# Autodesk Inventor assembly: BallBot
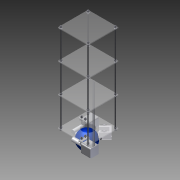
[picture p0: Inventor's stored thumbnail of the model, 180x180]
Saved by Autodesk Inventor 2012 (Build 160160000, 160)
## iProperties
Created: 2012-10-02
Part Number: BallBot
Document SubType Name: Assembly
Designer: agmlego
Author: agmlego
## Documents named in this file (16)
- H:\My Documents\Projects\BallBot\micro\CAD\BallBot.iam
- H:\My Documents\Projects\BallBot\micro\CAD\Platform.ipt
- H:\My Documents\Projects\BallBot\micro\CAD\Rod.ipt
- H:\My Documents\Projects\BallBot\micro\CAD\Ball.ipt
- \\derp\hdrives\agmeyer\My Documents\Inventor\Content Center Files\R2012\en-US\ANSI B 18.2.4.1 M(1)\ANSI B 18.2.4.1 M - M3 x 0.5Style 1.ipt
- H:\My Documents\Projects\BallBot\micro\CAD\211-13-01.ipt
- H:\My Documents\Projects\BallBot\micro\CAD\Roller.ipt
- \\derp\hdrives\agmeyer\My Documents\Inventor\Content Center Files\R2012\en-US\ANSI B18.3(08)\ANSI B18.3 - 4-48 UNF - 0.125(24).ipt
- H:\My Documents\Projects\BallBot\micro\CAD\Bottom_Platform.ipt
- H:\My Documents\Projects\BallBot\micro\CAD\Stepper_Bracket.ipt
- H:\My Documents\Projects\BallBot\micro\CAD\Tension_Housing.ipt
- H:\My Documents\Projects\BallBot\micro\CAD\Idler.ipt
- \\derp\hdrives\agmeyer\My Documents\Inventor\Content Center Files\R2012\en-US\ANSI B18.3.1M(6)\ANSI B18.3.1M - M3x0.5 x 35(1).ipt
- \\derp\hdrives\agmeyer\My Documents\Inventor\Content Center Files\R2012\en-US\ANSI B18.3.1M(6)\ANSI B18.3.1M - M2.5x0.45 x 10(1).ipt
- \\derp\hdrives\agmeyer\My Documents\Inventor\Content Center Files\R2012\en-US\ANSI B18.3.1M(6)\ANSI B18.3.1M - M3x0.5 x 10(1).ipt
- \\derp\hdrives\agmeyer\My Documents\Inventor\Content Center Files\R2012\en-US\ANSI B18.22 M\ANSI B18.22M - 3 N.ipt
## Components (103 placed, 15 different names)
1. Rod:1 — Mate:4, Mate:5, Mate:6, Mate:7, Mate:8, Mate:9, Mate:10, Mate:11, Mate:34, Mate:38, Mate:42, Mate:115, Mate:133, Mate:134, Mate:135, Mate:136, Mate:137, Mate:138, Mate:139, Mate:140, Flush:6, Flush:9
2. Rod:2 — Mate:1, Mate:3, Mate:12, Mate:13, Mate:14, Mate:15, Mate:16, Mate:17, Mate:35, Mate:39, Mate:43, Mate:114, Mate:145, Mate:146, Mate:147, Mate:148, Mate:149, Mate:150, Mate:153, Mate:154, Flush:5, Flush:11
3. Rod:3 — Mate:18, Mate:19, Mate:20, Mate:21, Mate:22, Mate:23, Mate:24, Mate:25, Mate:36, Mate:40, Mate:44, Mate:90, Mate:116, Mate:124, Mate:126, Mate:127, Mate:128, Mate:129, Mate:130, Mate:131, Mate:132, Flush:8, Flush:12
4. Rod:4 — Mate:26, Mate:27, Mate:28, Mate:29, Mate:30, Mate:31, Mate:32, Mate:33, Mate:37, Mate:41, Mate:45, Mate:117, Mate:155, Mate:156, Mate:157, Mate:158, Mate:159, Mate:160, Mate:161, Mate:162, Flush:7, Flush:10
5. Ball:1 — Tangent:5, Tangent:6, Tangent:8
6. Tension_Housing:1 — Mate:105, Mate:107, Mate:108, Mate:109, Insert:3, Insert:4
7. Idler:1 — Mate:107, Mate:108, Tangent:8
8. Forged Socket Head Cap Screw - Metric M3x0.5 x 35:1 — Insert:3
9. Hex Nut Metric M3 x 0.5:65 — Insert:4
10. 211-13-01:3 — Insert:2, Tangent:1, Tangent:2, Mate:97, Mate:98, Mate:99
11. Roller:1 — Insert:2, Mate:91, Mate:92, Tangent:6
12. Hexagon Socket Set Screw - Flat Point - Inch 4-48 UNF x 0.125:5 — Mate:91, Tangent:1
13. Hexagon Socket Set Screw - Flat Point - Inch 4-48 UNF x 0.125:7 — Mate:92, Tangent:2
14. Stepper_Bracket:1 — Mate:97, Mate:98, Mate:99, Mate:104, Insert:7, Insert:8, Mate:112, Mate:113, Insert:11, Insert:12
15. Forged Socket Head Cap Screw - Metric M2.5x0.45 x 10:3 — Insert:7
16. Forged Socket Head Cap Screw - Metric M2.5x0.45 x 10:4 — Insert:8
17. Forged Socket Head Cap Screw - Metric M3x0.5 x 10:2 — Insert:11, Mate:142
18. Forged Socket Head Cap Screw - Metric M3x0.5 x 10:4 — Insert:12, Mate:141
19. Hex Nut Metric M3 x 0.5:68 — Insert:21
20. Hex Nut Metric M3 x 0.5:69 — Insert:22
21. Plain Washer (Metric) 3 N:9 — Mate:141, Mate:227, Insert:22
22. Plain Washer (Metric) 3 N:10 — Mate:142, Mate:226, Insert:21
23. Stepper_Bracket:2 — Mate:100, Mate:101, Mate:102, Mate:103, Insert:5, Insert:6, Mate:110, Mate:111, Insert:9, Insert:10
24. 211-13-01:1 — Insert:1, Tangent:3, Tangent:4, Mate:100, Mate:101, Mate:102
25. Roller:2 — Insert:1, Mate:93, Mate:94, Tangent:5
26. Hexagon Socket Set Screw - Flat Point - Inch 4-48 UNF x 0.125:6 — Mate:94, Tangent:4
27. Hexagon Socket Set Screw - Flat Point - Inch 4-48 UNF x 0.125:8 — Mate:93, Tangent:3
28. Forged Socket Head Cap Screw - Metric M2.5x0.45 x 10:1 — Insert:5
29. Forged Socket Head Cap Screw - Metric M2.5x0.45 x 10:2 — Insert:6
30. Forged Socket Head Cap Screw - Metric M3x0.5 x 10:1 — Insert:9, Mate:143
31. Forged Socket Head Cap Screw - Metric M3x0.5 x 10:3 — Insert:10, Mate:144
32. Hex Nut Metric M3 x 0.5:66 — Insert:23
33. Hex Nut Metric M3 x 0.5:67 — Insert:24
34. Plain Washer (Metric) 3 N:11 — Mate:144, Mate:229, Insert:24
35. Plain Washer (Metric) 3 N:12 — Mate:143, Mate:228, Insert:23
36. Platform:3 — Mate:38, Mate:39, Mate:40, Mate:41, Mate:43, Mate:44, Mate:45, Mate:88, Mate:164, Mate:165, Mate:167, Mate:169, Mate:171, Mate:173, Mate:175, Mate:177
37. Hex Nut Metric M3 x 0.5:38 — Mate:31, Mate:172, Flush:7
38. Hex Nut Metric M3 x 0.5:40 — Mate:33, Mate:174
39. Hex Nut Metric M3 x 0.5:46 — Mate:9, Mate:170
40. Hex Nut Metric M3 x 0.5:47 — Mate:10, Mate:168, Flush:6
41. Hex Nut Metric M3 x 0.5:51 — Mate:12, Mate:166
42. Hex Nut Metric M3 x 0.5:56 — Mate:17, Mate:163, Flush:5
43. Hex Nut Metric M3 x 0.5:62 — Mate:23, Mate:176, Flush:8
44. Hex Nut Metric M3 x 0.5:63 — Mate:24, Mate:178
45. Plain Washer (Metric) 3 N:1 — Mate:132, Mate:177, Mate:178
46. Plain Washer (Metric) 3 N:2 — Mate:131, Mate:175, Mate:176
47. Plain Washer (Metric) 3 N:27 — Mate:133, Mate:167, Mate:168
48. Plain Washer (Metric) 3 N:28 — Mate:134, Mate:169, Mate:170
49. Plain Washer (Metric) 3 N:29 — Mate:153, Mate:163, Mate:164
50. Plain Washer (Metric) 3 N:30 — Mate:154, Mate:165, Mate:166
51. Plain Washer (Metric) 3 N:31 — Mate:155, Mate:171, Mate:172
52. Plain Washer (Metric) 3 N:32 — Mate:156, Mate:173, Mate:174
53. Platform:4 — Mate:42, Mate:88, Mate:89, Mate:90, Mate:180, Mate:181, Mate:184, Mate:185, Mate:188, Mate:189, Mate:192, Mate:193
54. Hex Nut Metric M3 x 0.5:35 — Mate:28, Mate:182
55. Hex Nut Metric M3 x 0.5:39 — Mate:32, Mate:179
56. Hex Nut Metric M3 x 0.5:41 — Mate:4, Mate:190
57. Hex Nut Metric M3 x 0.5:45 — Mate:8, Mate:187
58. Hex Nut Metric M3 x 0.5:53 — Mate:14, Mate:194
59. Hex Nut Metric M3 x 0.5:54 — Mate:15, Mate:191
60. Hex Nut Metric M3 x 0.5:60 — Mate:21, Mate:183
61. Hex Nut Metric M3 x 0.5:64 — Mate:25, Mate:186
62. Plain Washer (Metric) 3 N:3 — Mate:130, Mate:185, Mate:186
63. Plain Washer (Metric) 3 N:4 — Mate:129, Mate:183, Mate:184
64. Plain Washer (Metric) 3 N:21 — Mate:135, Mate:187, Mate:188
65. Plain Washer (Metric) 3 N:22 — Mate:136, Mate:189, Mate:190
66. Plain Washer (Metric) 3 N:23 — Mate:150, Mate:193, Mate:194
67. Plain Washer (Metric) 3 N:24 — Mate:149, Mate:191, Mate:192
68. Plain Washer (Metric) 3 N:33 — Mate:157, Mate:181, Mate:182
69. Plain Washer (Metric) 3 N:34 — Mate:158, Mate:179, Mate:180
70. Platform:2 — Mate:34, Mate:35, Mate:36, Mate:37, Mate:89, Mate:196, Mate:197, Mate:200, Mate:201, Mate:203, Mate:205, Mate:208, Mate:209
71. Hex Nut Metric M3 x 0.5:36 — Mate:29, Mate:210
72. Hex Nut Metric M3 x 0.5:37 — Mate:30, Mate:207
73. Hex Nut Metric M3 x 0.5:42 — Mate:5, Mate:199
74. Hex Nut Metric M3 x 0.5:48 — Mate:11, Mate:202
75. Hex Nut Metric M3 x 0.5:52 — Mate:13, Mate:198
76. Hex Nut Metric M3 x 0.5:55 — Mate:16, Mate:195
77. Hex Nut Metric M3 x 0.5:58 — Mate:19, Mate:206
78. Hex Nut Metric M3 x 0.5:59 — Mate:20, Mate:204
79. Plain Washer (Metric) 3 N:5 — Mate:128, Mate:205, Mate:206
80. Plain Washer (Metric) 3 N:6 — Mate:127, Mate:203, Mate:204
81. Plain Washer (Metric) 3 N:17 — Mate:147, Mate:197, Mate:198
82. Plain Washer (Metric) 3 N:18 — Mate:146, Mate:195, Mate:196
83. Plain Washer (Metric) 3 N:19 — Mate:137, Mate:199, Mate:200
84. Plain Washer (Metric) 3 N:20 — Mate:138, Mate:201, Mate:202
85. Plain Washer (Metric) 3 N:35 — Mate:159, Mate:209, Mate:210
86. Plain Washer (Metric) 3 N:36 — Mate:160, Mate:207, Mate:208
87. Bottom_Platform:1 — Mate:103, Mate:104, Mate:105, Mate:109, Mate:110, Mate:111, Mate:112, Mate:113, Mate:114, Mate:115, Mate:116, Mate:117, Mate:125, Mate:212, Mate:213, Mate:215, Mate:219, Mate:220, Mate:223, Mate:224, Mate:226, Mate:227, Mate:228, Mate:229
88. Hex Nut Metric M3 x 0.5:33 — Mate:26, Mate:214, Flush:10
89. Hex Nut Metric M3 x 0.5:34 — Mate:27, Mate:211
90. Hex Nut Metric M3 x 0.5:43 — Mate:6, Mate:225, Flush:9
91. Hex Nut Metric M3 x 0.5:44 — Mate:7, Mate:222
92. Hex Nut Metric M3 x 0.5:49 — Mate:1, Mate:221, Flush:11
93. Hex Nut Metric M3 x 0.5:50 — Mate:3, Mate:218
94. Hex Nut Metric M3 x 0.5:57 — Mate:18, Mate:216
95. Hex Nut Metric M3 x 0.5:61 — Mate:22, Mate:217, Flush:12
96. Plain Washer (Metric) 3 N:7 — Mate:126, Mate:215, Mate:216
97. Plain Washer (Metric) 3 N:8 — Mate:124, Mate:125, Mate:217
98. Plain Washer (Metric) 3 N:13 — Mate:148, Mate:218, Mate:219
99. Plain Washer (Metric) 3 N:14 — Mate:145, Mate:220, Mate:221
100. Plain Washer (Metric) 3 N:15 — Mate:139, Mate:222, Mate:223
101. Plain Washer (Metric) 3 N:16 — Mate:140, Mate:224, Mate:225
102. Plain Washer (Metric) 3 N:37 — Mate:161, Mate:211, Mate:212
103. Plain Washer (Metric) 3 N:38 — Mate:162, Mate:213, Mate:214
## Relationships (206: Mate 175, Insert 16, Flush 8, Tangent 7)
- Mate:1: Rod:2 ↔ Hex Nut Metric M3 x 0.5:49
- Mate:3: Rod:2 ↔ Hex Nut Metric M3 x 0.5:50
- Mate:4: Rod:1 ↔ Hex Nut Metric M3 x 0.5:41
- Mate:5: Rod:1 ↔ Hex Nut Metric M3 x 0.5:42
- Mate:6: Rod:1 ↔ Hex Nut Metric M3 x 0.5:43
- Mate:7: Rod:1 ↔ Hex Nut Metric M3 x 0.5:44
- Mate:8: Rod:1 ↔ Hex Nut Metric M3 x 0.5:45
- Mate:9: Rod:1 ↔ Hex Nut Metric M3 x 0.5:46
- Mate:10: Rod:1 ↔ Hex Nut Metric M3 x 0.5:47
- Mate:11: Rod:1 ↔ Hex Nut Metric M3 x 0.5:48
- Mate:12: Rod:2 ↔ Hex Nut Metric M3 x 0.5:51
- Mate:13: Rod:2 ↔ Hex Nut Metric M3 x 0.5:52
- Mate:14: Rod:2 ↔ Hex Nut Metric M3 x 0.5:53
- Mate:15: Rod:2 ↔ Hex Nut Metric M3 x 0.5:54
- Mate:16: Rod:2 ↔ Hex Nut Metric M3 x 0.5:55
- Mate:17: Rod:2 ↔ Hex Nut Metric M3 x 0.5:56
- Mate:18: Rod:3 ↔ Hex Nut Metric M3 x 0.5:57
- Mate:19: Rod:3 ↔ Hex Nut Metric M3 x 0.5:58
- Mate:20: Rod:3 ↔ Hex Nut Metric M3 x 0.5:59
- Mate:21: Rod:3 ↔ Hex Nut Metric M3 x 0.5:60
- Mate:22: Rod:3 ↔ Hex Nut Metric M3 x 0.5:61
- Mate:23: Rod:3 ↔ Hex Nut Metric M3 x 0.5:62
- Mate:24: Rod:3 ↔ Hex Nut Metric M3 x 0.5:63
- Mate:25: Rod:3 ↔ Hex Nut Metric M3 x 0.5:64
- Mate:26: Rod:4 ↔ Hex Nut Metric M3 x 0.5:33
- Mate:27: Rod:4 ↔ Hex Nut Metric M3 x 0.5:34
- Mate:28: Rod:4 ↔ Hex Nut Metric M3 x 0.5:35
- Mate:29: Rod:4 ↔ Hex Nut Metric M3 x 0.5:36
- Mate:30: Rod:4 ↔ Hex Nut Metric M3 x 0.5:37
- Mate:31: Rod:4 ↔ Hex Nut Metric M3 x 0.5:38
- Mate:32: Rod:4 ↔ Hex Nut Metric M3 x 0.5:39
- Mate:33: Rod:4 ↔ Hex Nut Metric M3 x 0.5:40
- Mate:34: Rod:1 ↔ Platform:2
- Mate:35: Rod:2 ↔ Platform:2
- Mate:36: Rod:3 ↔ Platform:2
- Mate:37: Rod:4 ↔ Platform:2
- Mate:38: Rod:1 ↔ Platform:3
- Mate:39: Rod:2 ↔ Platform:3
- Mate:40: Rod:3 ↔ Platform:3
- Mate:41: Rod:4 ↔ Platform:3
- Mate:42: Rod:1 ↔ Platform:4
- Mate:43: Rod:2 ↔ Platform:3
- Mate:44: Rod:3 ↔ Platform:3
- Mate:45: Rod:4 ↔ Platform:3
- Mate:88 (93.1 mm): Platform:3 ↔ Platform:4
- Mate:89 (93.1 mm): Platform:4 ↔ Platform:2
- Mate:90: Rod:3 ↔ Platform:4
- Insert:1: 211-13-01:1 ↔ Roller:2
- Insert:2: 211-13-01:3 ↔ Roller:1
- Mate:91: Roller:1 ↔ Hexagon Socket Set Screw - Flat Point - Inch 4-48 UNF x 0.125:5
- Mate:92: Roller:1 ↔ Hexagon Socket Set Screw - Flat Point - Inch 4-48 UNF x 0.125:7
- Mate:93: Roller:2 ↔ Hexagon Socket Set Screw - Flat Point - Inch 4-48 UNF x 0.125:8
- Mate:94: Roller:2 ↔ Hexagon Socket Set Screw - Flat Point - Inch 4-48 UNF x 0.125:6
- Tangent:1: 211-13-01:3 ↔ Hexagon Socket Set Screw - Flat Point - Inch 4-48 UNF x 0.125:5
- Tangent:2: 211-13-01:3 ↔ Hexagon Socket Set Screw - Flat Point - Inch 4-48 UNF x 0.125:7
- Tangent:3: 211-13-01:1 ↔ Hexagon Socket Set Screw - Flat Point - Inch 4-48 UNF x 0.125:8
- Tangent:4: 211-13-01:1 ↔ Hexagon Socket Set Screw - Flat Point - Inch 4-48 UNF x 0.125:6
- Tangent:5: Ball:1 ↔ Roller:2
- Tangent:6: Ball:1 ↔ Roller:1
- Mate:97: 211-13-01:3 ↔ Stepper_Bracket:1
- Mate:98: 211-13-01:3 ↔ Stepper_Bracket:1
- Mate:99: 211-13-01:3 ↔ Stepper_Bracket:1
- Mate:100: Stepper_Bracket:2 ↔ 211-13-01:1
- Mate:101: Stepper_Bracket:2 ↔ 211-13-01:1
- Mate:102: Stepper_Bracket:2 ↔ 211-13-01:1
- Mate:103: Stepper_Bracket:2 ↔ Bottom_Platform:1
- Mate:104: Stepper_Bracket:1 ↔ Bottom_Platform:1
- Mate:105: Tension_Housing:1 ↔ Bottom_Platform:1
- Mate:107: Tension_Housing:1 ↔ Idler:1
- Mate:108 (1 mm): Tension_Housing:1 ↔ Idler:1
- Tangent:8: Ball:1 ↔ Idler:1
- Mate:109 (0.05 mm): Tension_Housing:1 ↔ Bottom_Platform:1
- Insert:3: Tension_Housing:1 ↔ Forged Socket Head Cap Screw - Metric M3x0.5 x 35:1
- Insert:4: Tension_Housing:1 ↔ Hex Nut Metric M3 x 0.5:65
- Insert:5: Stepper_Bracket:2 ↔ Forged Socket Head Cap Screw - Metric M2.5x0.45 x 10:1
- Insert:6: Stepper_Bracket:2 ↔ Forged Socket Head Cap Screw - Metric M2.5x0.45 x 10:2
- Insert:7: Stepper_Bracket:1 ↔ Forged Socket Head Cap Screw - Metric M2.5x0.45 x 10:3
- Insert:8: Stepper_Bracket:1 ↔ Forged Socket Head Cap Screw - Metric M2.5x0.45 x 10:4
- Mate:110: Stepper_Bracket:2 ↔ Bottom_Platform:1
- Mate:111: Stepper_Bracket:2 ↔ Bottom_Platform:1
- Mate:112: Stepper_Bracket:1 ↔ Bottom_Platform:1
- Mate:113: Stepper_Bracket:1 ↔ Bottom_Platform:1
- Mate:114: Rod:2 ↔ Bottom_Platform:1
- Mate:115: Rod:1 ↔ Bottom_Platform:1
- Mate:116: Rod:3 ↔ Bottom_Platform:1
- Mate:117: Rod:4 ↔ Bottom_Platform:1
- Insert:9: Stepper_Bracket:2 ↔ Forged Socket Head Cap Screw - Metric M3x0.5 x 10:1
- Insert:10: Stepper_Bracket:2 ↔ Forged Socket Head Cap Screw - Metric M3x0.5 x 10:3
- Insert:11: Stepper_Bracket:1 ↔ Forged Socket Head Cap Screw - Metric M3x0.5 x 10:2
- Insert:12: Stepper_Bracket:1 ↔ Forged Socket Head Cap Screw - Metric M3x0.5 x 10:4
- Mate:124: Rod:3 ↔ Plain Washer (Metric) 3 N:8
- Mate:125: Bottom_Platform:1 ↔ Plain Washer (Metric) 3 N:8
- Mate:126: Rod:3 ↔ Plain Washer (Metric) 3 N:7
- Mate:127: Rod:3 ↔ Plain Washer (Metric) 3 N:6
- Mate:128: Rod:3 ↔ Plain Washer (Metric) 3 N:5
- Mate:129: Rod:3 ↔ Plain Washer (Metric) 3 N:4
- Mate:130: Rod:3 ↔ Plain Washer (Metric) 3 N:3
- Mate:131: Rod:3 ↔ Plain Washer (Metric) 3 N:2
- Mate:132: Rod:3 ↔ Plain Washer (Metric) 3 N:1
- Mate:133: Rod:1 ↔ Plain Washer (Metric) 3 N:27
- Mate:134: Rod:1 ↔ Plain Washer (Metric) 3 N:28
- Mate:135: Rod:1 ↔ Plain Washer (Metric) 3 N:21
- Mate:136: Rod:1 ↔ Plain Washer (Metric) 3 N:22
- Mate:137: Rod:1 ↔ Plain Washer (Metric) 3 N:19
- Mate:138: Rod:1 ↔ Plain Washer (Metric) 3 N:20
- Mate:139: Rod:1 ↔ Plain Washer (Metric) 3 N:15
- Mate:140: Rod:1 ↔ Plain Washer (Metric) 3 N:16
- Mate:141: Forged Socket Head Cap Screw - Metric M3x0.5 x 10:4 ↔ Plain Washer (Metric) 3 N:9
- Mate:142: Forged Socket Head Cap Screw - Metric M3x0.5 x 10:2 ↔ Plain Washer (Metric) 3 N:10
- Mate:143: Forged Socket Head Cap Screw - Metric M3x0.5 x 10:1 ↔ Plain Washer (Metric) 3 N:12
- Mate:144: Forged Socket Head Cap Screw - Metric M3x0.5 x 10:3 ↔ Plain Washer (Metric) 3 N:11
- Mate:145: Rod:2 ↔ Plain Washer (Metric) 3 N:14
- Mate:146: Rod:2 ↔ Plain Washer (Metric) 3 N:18
- Mate:147: Rod:2 ↔ Plain Washer (Metric) 3 N:17
- Mate:148: Rod:2 ↔ Plain Washer (Metric) 3 N:13
- Mate:149: Rod:2 ↔ Plain Washer (Metric) 3 N:24
- Mate:150: Rod:2 ↔ Plain Washer (Metric) 3 N:23
- Mate:153: Rod:2 ↔ Plain Washer (Metric) 3 N:29
- Mate:154: Rod:2 ↔ Plain Washer (Metric) 3 N:30
- Mate:155: Rod:4 ↔ Plain Washer (Metric) 3 N:31
- Mate:156: Rod:4 ↔ Plain Washer (Metric) 3 N:32
- Mate:157: Rod:4 ↔ Plain Washer (Metric) 3 N:33
- Mate:158: Rod:4 ↔ Plain Washer (Metric) 3 N:34
- Mate:159: Rod:4 ↔ Plain Washer (Metric) 3 N:35
- Mate:160: Rod:4 ↔ Plain Washer (Metric) 3 N:36
- Mate:161: Rod:4 ↔ Plain Washer (Metric) 3 N:37
- Mate:162: Rod:4 ↔ Plain Washer (Metric) 3 N:38
- Mate:163: Hex Nut Metric M3 x 0.5:56 ↔ Plain Washer (Metric) 3 N:29
- Mate:164: Platform:3 ↔ Plain Washer (Metric) 3 N:29
- Mate:165: Platform:3 ↔ Plain Washer (Metric) 3 N:30
- Mate:166: Hex Nut Metric M3 x 0.5:51 ↔ Plain Washer (Metric) 3 N:30
- Mate:167: Platform:3 ↔ Plain Washer (Metric) 3 N:27
- Mate:168: Hex Nut Metric M3 x 0.5:47 ↔ Plain Washer (Metric) 3 N:27
- Mate:169: Platform:3 ↔ Plain Washer (Metric) 3 N:28
- Mate:170: Hex Nut Metric M3 x 0.5:46 ↔ Plain Washer (Metric) 3 N:28
- Mate:171: Platform:3 ↔ Plain Washer (Metric) 3 N:31
- Mate:172: Hex Nut Metric M3 x 0.5:38 ↔ Plain Washer (Metric) 3 N:31
- Mate:173: Platform:3 ↔ Plain Washer (Metric) 3 N:32
- Mate:174: Hex Nut Metric M3 x 0.5:40 ↔ Plain Washer (Metric) 3 N:32
- Mate:175: Platform:3 ↔ Plain Washer (Metric) 3 N:2
- Mate:176: Hex Nut Metric M3 x 0.5:62 ↔ Plain Washer (Metric) 3 N:2
- Mate:177: Platform:3 ↔ Plain Washer (Metric) 3 N:1
- Mate:178: Hex Nut Metric M3 x 0.5:63 ↔ Plain Washer (Metric) 3 N:1
- Flush:5 (1 mm): Rod:2 ↔ Hex Nut Metric M3 x 0.5:56
- Flush:6 (-1 mm): Rod:1 ↔ Hex Nut Metric M3 x 0.5:47
- Flush:7 (1 mm): Rod:4 ↔ Hex Nut Metric M3 x 0.5:38
- Flush:8 (1 mm): Rod:3 ↔ Hex Nut Metric M3 x 0.5:62
- Mate:179: Hex Nut Metric M3 x 0.5:39 ↔ Plain Washer (Metric) 3 N:34
- Mate:180: Platform:4 ↔ Plain Washer (Metric) 3 N:34
- Mate:181: Platform:4 ↔ Plain Washer (Metric) 3 N:33
- Mate:182: Hex Nut Metric M3 x 0.5:35 ↔ Plain Washer (Metric) 3 N:33
- Mate:183: Hex Nut Metric M3 x 0.5:60 ↔ Plain Washer (Metric) 3 N:4
- Mate:184: Platform:4 ↔ Plain Washer (Metric) 3 N:4
- Mate:185: Platform:4 ↔ Plain Washer (Metric) 3 N:3
- Mate:186: Hex Nut Metric M3 x 0.5:64 ↔ Plain Washer (Metric) 3 N:3
- Mate:187: Hex Nut Metric M3 x 0.5:45 ↔ Plain Washer (Metric) 3 N:21
- Mate:188: Platform:4 ↔ Plain Washer (Metric) 3 N:21
- Mate:189: Platform:4 ↔ Plain Washer (Metric) 3 N:22
- Mate:190: Hex Nut Metric M3 x 0.5:41 ↔ Plain Washer (Metric) 3 N:22
- Mate:191: Hex Nut Metric M3 x 0.5:54 ↔ Plain Washer (Metric) 3 N:24
- Mate:192: Platform:4 ↔ Plain Washer (Metric) 3 N:24
- Mate:193: Platform:4 ↔ Plain Washer (Metric) 3 N:23
- Mate:194: Hex Nut Metric M3 x 0.5:53 ↔ Plain Washer (Metric) 3 N:23
- Mate:195: Hex Nut Metric M3 x 0.5:55 ↔ Plain Washer (Metric) 3 N:18
- Mate:196: Platform:2 ↔ Plain Washer (Metric) 3 N:18
- Mate:197: Platform:2 ↔ Plain Washer (Metric) 3 N:17
- Mate:198: Hex Nut Metric M3 x 0.5:52 ↔ Plain Washer (Metric) 3 N:17
- Mate:199: Hex Nut Metric M3 x 0.5:42 ↔ Plain Washer (Metric) 3 N:19
- Mate:200: Platform:2 ↔ Plain Washer (Metric) 3 N:19
- Mate:201: Platform:2 ↔ Plain Washer (Metric) 3 N:20
- Mate:202: Hex Nut Metric M3 x 0.5:48 ↔ Plain Washer (Metric) 3 N:20
- Mate:203: Platform:2 ↔ Plain Washer (Metric) 3 N:6
- Mate:204: Hex Nut Metric M3 x 0.5:59 ↔ Plain Washer (Metric) 3 N:6
- Mate:205: Platform:2 ↔ Plain Washer (Metric) 3 N:5
- Mate:206: Hex Nut Metric M3 x 0.5:58 ↔ Plain Washer (Metric) 3 N:5
- Mate:207: Hex Nut Metric M3 x 0.5:37 ↔ Plain Washer (Metric) 3 N:36
- Mate:208: Platform:2 ↔ Plain Washer (Metric) 3 N:36
- Mate:209: Platform:2 ↔ Plain Washer (Metric) 3 N:35
- Mate:210: Hex Nut Metric M3 x 0.5:36 ↔ Plain Washer (Metric) 3 N:35
- Mate:211: Hex Nut Metric M3 x 0.5:34 ↔ Plain Washer (Metric) 3 N:37
- Mate:212: Bottom_Platform:1 ↔ Plain Washer (Metric) 3 N:37
- Mate:213: Bottom_Platform:1 ↔ Plain Washer (Metric) 3 N:38
- Mate:214: Hex Nut Metric M3 x 0.5:33 ↔ Plain Washer (Metric) 3 N:38
- Mate:215: Bottom_Platform:1 ↔ Plain Washer (Metric) 3 N:7
- Mate:216: Hex Nut Metric M3 x 0.5:57 ↔ Plain Washer (Metric) 3 N:7
- Mate:217: Hex Nut Metric M3 x 0.5:61 ↔ Plain Washer (Metric) 3 N:8
- Mate:218: Hex Nut Metric M3 x 0.5:50 ↔ Plain Washer (Metric) 3 N:13
- Mate:219: Bottom_Platform:1 ↔ Plain Washer (Metric) 3 N:13
- Mate:220: Bottom_Platform:1 ↔ Plain Washer (Metric) 3 N:14
- Mate:221: Hex Nut Metric M3 x 0.5:49 ↔ Plain Washer (Metric) 3 N:14
- Mate:222: Hex Nut Metric M3 x 0.5:44 ↔ Plain Washer (Metric) 3 N:15
- Mate:223: Bottom_Platform:1 ↔ Plain Washer (Metric) 3 N:15
- Mate:224: Bottom_Platform:1 ↔ Plain Washer (Metric) 3 N:16
- Mate:225: Hex Nut Metric M3 x 0.5:43 ↔ Plain Washer (Metric) 3 N:16
- Flush:9 (1 mm): Rod:1 ↔ Hex Nut Metric M3 x 0.5:43
- Flush:10 (1 mm): Rod:4 ↔ Hex Nut Metric M3 x 0.5:33
- Flush:11 (1 mm): Rod:2 ↔ Hex Nut Metric M3 x 0.5:49
- Flush:12 (1 mm): Rod:3 ↔ Hex Nut Metric M3 x 0.5:61
- Mate:226: Plain Washer (Metric) 3 N:10 ↔ Bottom_Platform:1
- Mate:227: Plain Washer (Metric) 3 N:9 ↔ Bottom_Platform:1
- Insert:21: Hex Nut Metric M3 x 0.5:68 ↔ Plain Washer (Metric) 3 N:10
- Insert:22: Hex Nut Metric M3 x 0.5:69 ↔ Plain Washer (Metric) 3 N:9
- Mate:228: Plain Washer (Metric) 3 N:12 ↔ Bottom_Platform:1
- Mate:229: Plain Washer (Metric) 3 N:11 ↔ Bottom_Platform:1
- Insert:23: Hex Nut Metric M3 x 0.5:66 ↔ Plain Washer (Metric) 3 N:12
- Insert:24: Hex Nut Metric M3 x 0.5:67 ↔ Plain Washer (Metric) 3 N:11
